# Autodesk Inventor assembly: fc18-144
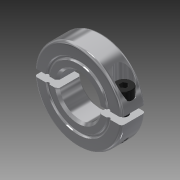
[picture p0: Inventor's stored thumbnail of the model, 180x180]
Saved by Autodesk Inventor 2018 (Build 220112000, 112)
## iProperties
Category: Miscellaneous
Company: Autodesk Inc.
Created: 2017-11-27
Part Number: fc18-144
Document SubType Name: Assembly
Designer: Autodesk Inc.
Catalog Web Link: https://www.ruland.com/ENSP20-6-A.html
Vendor: Ruland
Stock Number: ENSP20-6-A
Author: Autodesk Inc.
Keywords: FIRST Choice
## Documents named in this file (3)
- F:\FIRST 2018\FIRST 2018 FirstChoice\fc18-144_ShaftCollar.iam
- F:\FIRST 2018\FIRST 2018 FirstChoice\Parts\MISC_Collar_ENSP20-6-A.ipt
- F:\FIRST 2018\FIRST 2018 FirstChoice\Parts\ISO 4762 - M2 x 6ISO.ipt
## Components (3 placed, 2 different names)
1. MISC_Collar_ENSP20-6-A:1 — Insert:1, Insert:2
2. ISO 4762 M2 x 6:1 — Insert:1
3. ISO 4762 M2 x 6:2 — Insert:2
## Relationships (2: Insert 2)
- Insert:1: MISC_Collar_ENSP20-6-A:1 ↔ ISO 4762 M2 x 6:1
- Insert:2: MISC_Collar_ENSP20-6-A:1 ↔ ISO 4762 M2 x 6:2
